# Autodesk Inventor assembly: 4901_robot
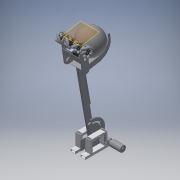
[picture p0: Inventor's stored thumbnail of the model, 180x180]
Saved by Autodesk Inventor 2016 (Build 200138000, 138)
## iProperties
Created: 2016-02-09
Part Number: 4901_robot
Document SubType Name: Assembly
Designer: Mentor1102
Sending System: CREO PARAMETRIC BY PTC INC, 2014440
Preprocessor: CREO PARAMETRIC BY PTC INC, 2014440
Title: ROBOT2_ASM
Author: folkj_000
Revision Number: 32LAST_VERSION
## Documents named in this file (11)
- C:\Users\Mentor1102\Desktop\4901 CAD\RobotArm\4901_robot.iam
- C:\Users\Mentor1102\Desktop\4901 CAD\RobotArm\BASE_ARM_SUPPORTS.ipt
- C:\Users\Mentor1102\Desktop\4901 CAD\RobotArm\VERTICAL_ARM_SUPPORTS.ipt
- C:\Users\Mentor1102\Desktop\4901 CAD\RobotArm\TOP_SUPPORTS_ARM.ipt
- C:\Users\Mentor1102\Desktop\4901 CAD\RobotArm\CIM_VERSAPLANETARY_ASM.iam
- C:\Users\Mentor1102\Desktop\4901 CAD\RobotArm\SMALL_GEAR.ipt
- C:\Users\Mentor1102\Desktop\4901 CAD\RobotArm\ARMSHAFT.ipt
- C:\Users\Mentor1102\Desktop\4901 CAD\RobotArm\PLATE_LOCK.ipt
- C:\Users\Mentor1102\Desktop\4901 CAD\RobotArm\CYLINDER.ipt
- C:\Users\Mentor1102\Desktop\4901 CAD\RobotArm\SHAFT_LOCK.ipt
- C:\Users\Mentor1102\Desktop\4901 CAD\Intake Claw Prototype.iam
## Components (17 placed, 17 different names)
1. 184
2. 185
3. 186
4. 187
5. 188 — Angle:1
6. 189
7. 190
8. 191 — Insert:2
9. 292 [sub-assembly]
10. 293
11. 294 — Insert:1, Insert:2
12. 295
13. 296
14. 297
15. 298
16. 299
17. Intake Claw Prototype:1 [sub-assembly] — Insert:1, Angle:1
## Relationships (3: Insert 2, Angle 1)
- Insert:1 (-101.6 mm): 294 ↔ Intake Claw Prototype:1
- Insert:2 (-165.1 mm): 191 ↔ 294
- Angle:1 (-10 deg): 188 ↔ Intake Claw Prototype:1
